# Autodesk Inventor assembly: bumper test
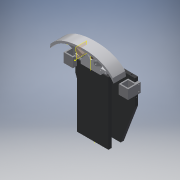
[picture p0: Inventor's stored thumbnail of the model, 180x180]
Saved by Autodesk Inventor 2016 (Build 200138000, 138)
## iProperties
Created: 2015-09-30
Part Number: bumper test
Document SubType Name: Assembly
Designer: Jesse Stevenson
Author: Jesse Stevenson
## Documents named in this file (10)
- C:\Users\Jesse Stevenson\Desktop\E-121-Design\bumper test.iam
- C:\Users\Jesse Stevenson\Desktop\E-121-Design\top.ipt
- C:\Users\Jesse Stevenson\Desktop\E-121-Design\bottom.ipt
- C:\Users\Jesse Stevenson\Desktop\E-121-Design\Microswitch_-_Omron_D2SW-P2L2T.iam
- C:\Users\Jesse Stevenson\Desktop\E-121-Design\bumper lever support.ipt
- C:\Users\Jesse Stevenson\Desktop\E-121-Design\lever2.ipt
- C:\Users\Jesse Stevenson\Desktop\E-121-Design\bumper.ipt
- C:\Users\Jesse Stevenson\Desktop\E-121-Design\lever2-flipped.ipt
- C:\Users\Jesse Stevenson\Desktop\E-121-Design\light sensor mounts\Light sensor shield 2.ipt
- C:\Users\Jesse Stevenson\Desktop\E-121-Design\light sensor mounts\Light sensor shield 2_MIR.ipt
## Components (10 placed, 9 different names)
1. top:1 — Flush:1, Mate:1, Mate:2, Mate:32, Flush:2, Flush:3, Flush:4, Mate:33, Mate:34
2. bottom:1 — Flush:1, Mate:1, Mate:3, Mate:20, Angle:2, Mate:21
3. Microswitch_-_Omron_D2SW-P2L2T:1 [sub-assembly] — Mate:27, Angle:4, Mate:28
4. Microswitch_-_Omron_D2SW-P2L2T:2 [sub-assembly] — Mate:25, Angle:3, Mate:26
5. bumper lever support:1 — Mate:20, Angle:2, Mate:21, Mate:22, Mate:23, Mate:24, Mate:25, Angle:3, Mate:26, Mate:27, Angle:4, Mate:28
6. bumper:1 — Mate:8, Mate:9, Mate:15, Mate:29, Mate:30
7. lever2-flipped:1 — Mate:15, Mate:23, Mate:29, Mate:30
8. lever2:2 — Mate:8, Mate:9, Mate:22, Mate:24
9. Light sensor shield 2:1 — Mate:32, Flush:2, Flush:3
10. Light sensor shield 2_MIR:1 — Flush:4, Mate:33, Mate:34
## Relationships (28: Mate 21, Flush 4, Angle 3)
- Flush:1: top:1 ↔ bottom:1
- Mate:1 (18.923 mm): top:1 ↔ bottom:1
- Mate:2: top:1
- Mate:3: bottom:1
- Mate:4 (25.273 mm)
- Mate:8: bumper:1 ↔ lever2:2
- Mate:9: bumper:1 ↔ lever2:2
- Mate:15: bumper:1 ↔ lever2-flipped:1
- Mate:20: bottom:1 ↔ bumper lever support:1
- Angle:2 (0 deg): bottom:1 ↔ bumper lever support:1
- Mate:21: bottom:1 ↔ bumper lever support:1
- Mate:22: bumper lever support:1 ↔ lever2:2
- Mate:23: bumper lever support:1 ↔ lever2-flipped:1
- Mate:24: bumper lever support:1 ↔ lever2:2
- Mate:25: Microswitch_-_Omron_D2SW-P2L2T:2 ↔ bumper lever support:1
- Angle:3 (0 deg): Microswitch_-_Omron_D2SW-P2L2T:2 ↔ bumper lever support:1
- Mate:26: Microswitch_-_Omron_D2SW-P2L2T:2 ↔ bumper lever support:1
- Mate:27: Microswitch_-_Omron_D2SW-P2L2T:1 ↔ bumper lever support:1
- Angle:4 (0 deg): Microswitch_-_Omron_D2SW-P2L2T:1 ↔ bumper lever support:1
- Mate:28: Microswitch_-_Omron_D2SW-P2L2T:1 ↔ bumper lever support:1
- Mate:29: bumper:1 ↔ lever2-flipped:1
- Mate:30: bumper:1 ↔ lever2-flipped:1
- Mate:32: top:1 ↔ Light sensor shield 2:1
- Flush:2 (-5.08 mm): top:1 ↔ Light sensor shield 2:1
- Flush:3 (-7.3914 mm): top:1 ↔ Light sensor shield 2:1
- Flush:4: top:1 ↔ Light sensor shield 2_MIR:1
- Mate:33: top:1 ↔ Light sensor shield 2_MIR:1
- Mate:34: top:1 ↔ Light sensor shield 2_MIR:1
